# Autodesk Inventor assembly: PaddleCollection
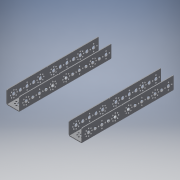
[picture p0: Inventor's stored thumbnail of the model, 180x180]
Saved by Autodesk Inventor 2019 (Build 230136000, 136)
## iProperties
Created: 2018-10-18
Part Number: PaddleCollection
Document SubType Name: Assembly
Designer: User
Author: User
## Documents named in this file (4)
- C:\Robotics\CAD\2018-19_CAD\Collection\PaddleCollection.iam
- C:\Robotics\CAD\COTSParts\Tetrix\Tetrix channel 124 mm.ipt
- C:\Robotics\CAD\COTSParts\Tetrix\Tetrix channel 96mm.ipt
- C:\Robotics\CAD\COTSParts\Tetrix\39274_txm-flat64mmx27mm.ipt
## Components (6 placed, 3 different names)
1. Tetrix channel 124 mm:1 — Insert:3
2. Tetrix channel 124 mm:2 — Insert:1
3. Tetrix channel 96mm:1 — Insert:4
4. Tetrix channel 96mm:2 — Insert:2
5. 39274_txm-flat64mmx27mm:1 — Insert:3, Insert:4
6. 39274_txm-flat64mmx27mm:2 — Insert:1, Insert:2
## Relationships (4: Insert 4)
- Insert:1: Tetrix channel 124 mm:2 ↔ 39274_txm-flat64mmx27mm:2
- Insert:2: Tetrix channel 96mm:2 ↔ 39274_txm-flat64mmx27mm:2
- Insert:3: Tetrix channel 124 mm:1 ↔ 39274_txm-flat64mmx27mm:1
- Insert:4: Tetrix channel 96mm:1 ↔ 39274_txm-flat64mmx27mm:1
